# Autodesk Inventor assembly: keyswitch_cherrymx
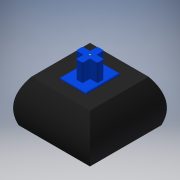
[picture p0: Inventor's stored thumbnail of the model, 180x180]
Saved by Autodesk Inventor 2016 (Build 200138000, 138)
## iProperties
Created: 2016-12-08
Part Number: keyswitch_cherrymx
Document SubType Name: Assembly
Designer: Cemra JC
Author: Cemra JC
## Documents named in this file (3)
- J:\The Files\The Software Files\Projects\stenotoppers\cherrymx\base-model\keyswitch_cherrymx.iam
- J:\The Files\The Software Files\Projects\stenotoppers\cherrymx\base-model\keyswitch-base_cherrymx.ipt
- J:\The Files\The Software Files\Projects\stenotoppers\cherrymx\base-model\keyswitch-pole_cherrymx.ipt
## Components (2 placed, 2 different names)
1. keyswitch-base_cherrymx:1 — Slider:1
2. keyswitch-pole_cherrymx:1 — Slider:1
## Relationships (1: TranslationJoint 1)
- Slider:1 [TranslationJoint]: keyswitch-base_cherrymx:1 ↔ keyswitch-pole_cherrymx:1
